# Autodesk Inventor assembly: AttendAssemble
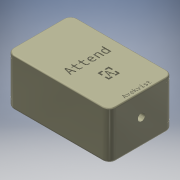
[picture p0: Inventor's stored thumbnail of the model, 180x180]
Saved by Autodesk Inventor 2019 (Build 230136000, 136)
## iProperties
Created: 2018-11-13
Part Number: AttendAssemble
Document SubType Name: Assembly
Designer: hampu
Author: hampu
## Documents named in this file (4)
- D:\OneDrive\Projects\Attend\HardwareDesign\AttendAssemble.iam
- D:\OneDrive\Projects\Attend\HardwareDesign\AttendBottom.ipt
- D:\OneDrive\Projects\Attend\HardwareDesign\AttendMiddle.ipt
- D:\OneDrive\Projects\Attend\HardwareDesign\AttendTop.ipt
## Components (3 placed, 3 different names)
1. AttendBottom:1 — Rigid:1
2. AttendMiddle:1 — Rigid:1, Rigid:2
3. AttendTop:1 — Rigid:2
## Relationships (2: WeldJoint 2)
- Rigid:1 [WeldJoint]: AttendBottom:1 ↔ AttendMiddle:1
- Rigid:2 [WeldJoint]: AttendMiddle:1 ↔ AttendTop:1
